# Autodesk Inventor assembly: 01-03-01 Zange Links
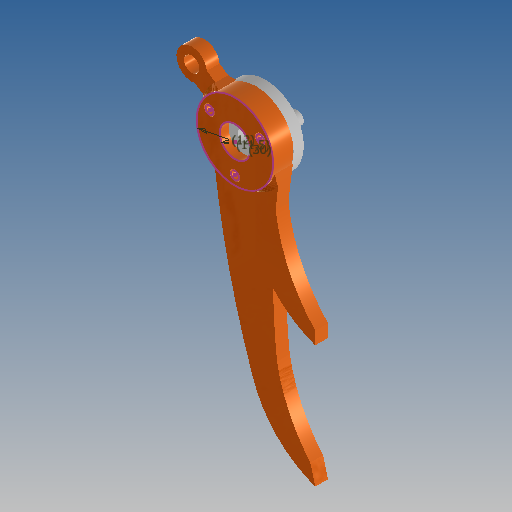
[picture p0: Inventor's stored thumbnail of the model, 512x512]
Saved by Autodesk Inventor 2026.2 (Build 302298000, 298)
## iProperties
Created: 2026-01-31
Part Number: 01-03-01 Zange Links
Document SubType Name: Assembly
Designer: Schally
Author: Schally
## Documents named in this file (5)
- E:\06 Carologistics\02 Zeichnungen Greifer System\Gripper Version 2 speziell deutsche Meisterschaft\01-03-01 Zange Links.iam
- E:\06 Carologistics\02 Zeichnungen Greifer System\Gripper Version 2 speziell deutsche Meisterschaft\01-03-01-01 Zeichnung Zange links unten.ipt
- E:\06 Carologistics\02 Zeichnungen Greifer System\Gripper Version 2 speziell deutsche Meisterschaft\01-03-01-02 Zeichnung Zange links oben.ipt
- E:\06 Carologistics\02 Zeichnungen Greifer System\Gripper Version 2 speziell deutsche Meisterschaft\01-03-01-03 Schraube kl.ipt
- E:\06 Carologistics\02 Zeichnungen Greifer System\Gripper Version 2 speziell deutsche Meisterschaft\01-03-01-04 Kugellager Tarik.ipt
## Components (6 placed, 4 different names)
1. 01-03-01-01 Zeichnung Zange links unten:1 — Passend:1, Passend:2, Passend:3, Passend:4
2. 01-03-01-02 Zeichnung Zange links oben:1 — Passend:1, Passend:2, Einfügen:1, Einfügen:2, Einfügen:3
3. 01-03-01-03 Schraube kl:1 — Einfügen:1
4. 01-03-01-03 Schraube kl:2 — Einfügen:2
5. 01-03-01-03 Schraube kl:3 — Einfügen:3
6. 01-03-01-04 Kugellager Tarik:1 — Passend:3, Passend:4
## Relationships (7: Mate 4, Insert 3)
- Passend:1 [Mate]: 01-03-01-01 Zeichnung Zange links unten:1 ↔ 01-03-01-02 Zeichnung Zange links oben:1
- Passend:2 [Mate]: 01-03-01-01 Zeichnung Zange links unten:1 ↔ 01-03-01-02 Zeichnung Zange links oben:1
- Einfügen:1 [Insert]: 01-03-01-02 Zeichnung Zange links oben:1 ↔ 01-03-01-03 Schraube kl:1
- Einfügen:2 [Insert]: 01-03-01-02 Zeichnung Zange links oben:1 ↔ 01-03-01-03 Schraube kl:2
- Einfügen:3 [Insert]: 01-03-01-02 Zeichnung Zange links oben:1 ↔ 01-03-01-03 Schraube kl:3
- Passend:3 [Mate]: 01-03-01-01 Zeichnung Zange links unten:1 ↔ 01-03-01-04 Kugellager Tarik:1
- Passend:4 [Mate]: 01-03-01-01 Zeichnung Zange links unten:1 ↔ 01-03-01-04 Kugellager Tarik:1
